# Autodesk Inventor assembly: derive_rod_v7
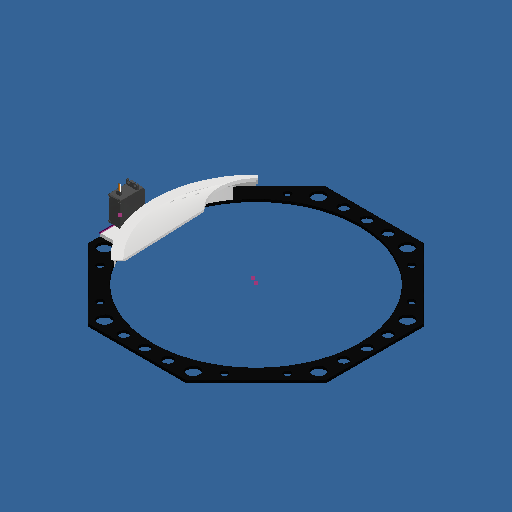
[picture p0: Inventor's stored thumbnail of the model, 512x512]
Saved by Autodesk Inventor 2026.2 (Build 302298000, 298)
## iProperties
Created: 2026-01-13
Part Number: derive_rod_v7
Document SubType Name: Assembly
Designer: Thoma
Author: Thoma
## Documents named in this file (5)
- C:\Users\Thoma\OneDrive\Desktop\dir\telescope_cover\cover\derive_rod_v7.iam
- C:\Users\Thoma\OneDrive\Desktop\dir\telescope_cover\telescope\version_3\Telescope_End.ipt
- C:\Users\Thoma\OneDrive\Desktop\dir\telescope_cover\cover\Cover_Upper_v3.ipt
- C:\Users\Thoma\OneDrive\Desktop\dir\telescope_cover\cover\Base_Plate_v2.ipt
- C:\Users\Thoma\OneDrive\Desktop\dir\telescope_cover\servo\DSS-M15S Servo.ipt
## Components (4 placed, 4 different names)
1. Telescope_End:1 — Mate:1, Mate:2, Angle:4, Mate:3, Mate:4, Mate:5, Flush:1
2. Cover_Upper_v3:1 — Mate:1, Mate:2, Angle:4
3. Base_Plate_v2:1 — Mate:3, Mate:4, Mate:5, Mate:6, Flush:8
4. DSS-M15S Servo:1 — Mate:6, Flush:1, Flush:8
## Relationships (9: Mate 6, Flush 2, Angle 1)
- Mate:1: Telescope_End:1 ↔ Cover_Upper_v3:1
- Mate:2 (1.977 mm): Telescope_End:1 ↔ Cover_Upper_v3:1
- Angle:4 (45 deg): Telescope_End:1 ↔ Cover_Upper_v3:1
- Mate:3: Telescope_End:1 ↔ Base_Plate_v2:1
- Mate:4: Telescope_End:1 ↔ Base_Plate_v2:1
- Mate:5: Telescope_End:1 ↔ Base_Plate_v2:1
- Mate:6 (7 mm): Base_Plate_v2:1 ↔ DSS-M15S Servo:1
- Flush:1: Telescope_End:1 ↔ DSS-M15S Servo:1
- Flush:8 (13.475 mm): Base_Plate_v2:1 ↔ DSS-M15S Servo:1
